# Autodesk Inventor assembly: CM_Assembly
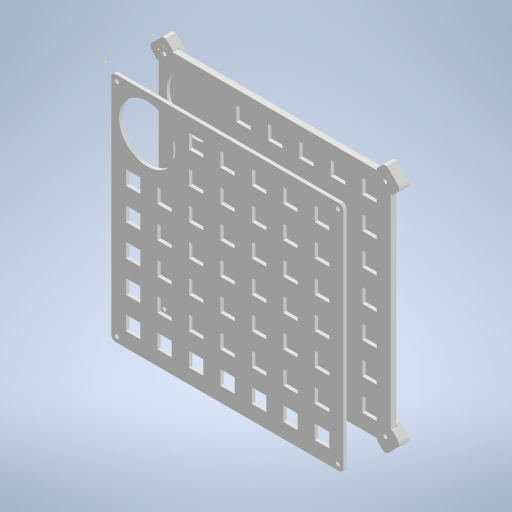
[picture p0: Inventor's stored thumbnail of the model, 512x512]
Saved by Autodesk Inventor 2023 (Build 270158000, 158)
## iProperties
Created: 2023-09-28
Part Number: CM_Assembly
Document SubType Name: Assembly
Designer: au323799
Author: au323799
## Documents named in this file (4)
- C:\Users\au323799\OneDrive - Aarhus Universitet\A_Articles\ASM_AuNP\3-Automation\Figures\CAD\CM_Assembly.iam
- C:\Users\au323799\OneDrive - Aarhus Universitet\A_Articles\ASM_AuNP\3-Automation\Figures\CAD\CM_bottom.ipt
- C:\Users\au323799\OneDrive - Aarhus Universitet\A_Articles\ASM_AuNP\3-Automation\Figures\CAD\CM_corner_piece.ipt
- C:\Users\au323799\OneDrive - Aarhus Universitet\A_Articles\ASM_AuNP\3-Automation\Figures\CAD\CM_top.ipt
## Components (6 placed, 3 different names)
1. CM_bottom:1 — Rotational:1, Rotational:2, Rotational:3, Rotational:4, Mate:1, Mate:2, Mate:3, Mate:4, Rotational:5, Rotational:6
2. CM_corner_piece:1 — Rotational:1, Mate:1
3. CM_corner_piece:2 — Rotational:2, Mate:2
4. CM_corner_piece:3 — Rotational:4, Mate:4
5. CM_corner_piece:4 — Rotational:3, Mate:3
6. CM_top:1 — Rotational:5, Rotational:6
## Relationships (10: RevoluteJoint 6, Mate 4)
- Rotational:1 [RevoluteJoint] (-10 mm): CM_bottom:1 ↔ CM_corner_piece:1
- Rotational:2 [RevoluteJoint] (-10 mm): CM_bottom:1 ↔ CM_corner_piece:2
- Rotational:3 [RevoluteJoint] (-10 mm): CM_bottom:1 ↔ CM_corner_piece:4
- Rotational:4 [RevoluteJoint] (-10 mm): CM_bottom:1 ↔ CM_corner_piece:3
- Mate:1: CM_bottom:1 ↔ CM_corner_piece:1
- Mate:2: CM_bottom:1 ↔ CM_corner_piece:2
- Mate:3: CM_bottom:1 ↔ CM_corner_piece:4
- Mate:4: CM_bottom:1 ↔ CM_corner_piece:3
- Rotational:5 [RevoluteJoint] (-40 mm): CM_bottom:1 ↔ CM_top:1
- Rotational:6 [RevoluteJoint] (-40 mm): CM_bottom:1 ↔ CM_top:1
